# Autodesk Inventor assembly: 200-60-DIFFERENTIAL-BAR-01
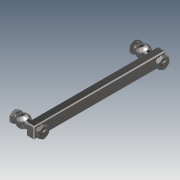
[picture p0: Inventor's stored thumbnail of the model, 180x180]
Saved by Autodesk Inventor 2018.2 (Build 222227000, 227)
## iProperties
Manager: feesmrt
Company: FRANCOR
Part Number: 200-60-DIFFERENTIAL-BAR-01
Project: Rescue Robot
Cost Center: -
Material: Generisch
Document SubType Name: Assembly
Designer: feesmrt
Engineer: feesmrt
Authority: feesmrt
Description: Differential Verbinder ASM
Stock Number: 200-60-DIFFERENTIAL-BAR-01
Subject: Rescue Robot
Author: feesmrt
Revision Number: 1
Title: Differential Verbinder ASM
## Documents named in this file (6)
- D:\Programmierung\FRANC0R\CAD\02-Rocker-Bogie-Robot\200-ROCKER-BOGIE\200-60-DIFFERENTIAL\200-60-DIFFERENTIAL-BAR-01.iam
- D:\Programmierung\FRANC0R\CAD\02-Rocker-Bogie-Robot\200-ROCKER-BOGIE\200-60-DIFFERENTIAL\200-60-DIFFERENTIAL-BAR-05.ipt
- D:\Programmierung\FRANC0R\CAD\02-Rocker-Bogie-Robot\200-ROCKER-BOGIE\200-60-DIFFERENTIAL\200-60-DIFFERENTIAL-BAR-04.ipt
- D:\Programmierung\FRANC0R\CAD\02-Rocker-Bogie-Robot\900-COMPONENTS\900-70-ANGLE-JOINTS\900-70-ANGLE-JOINT-DIN648-M8-2.ipt
- D:\Programmierung\FRANC0R\CAD\02-Rocker-Bogie-Robot\900-COMPONENTS\900-80-WASHERS\900-80-WASHERS-ISO8738-8.ipt
- D:\Programmierung\FRANC0R\CAD\02-Rocker-Bogie-Robot\900-COMPONENTS\900-41-NUTS\900-41-NUTS-ISO4035-M8.ipt
## Components (13 placed, 5 different names)
1. 200-60-DIFFERENTIAL-BAR-05:1 — Passend:1, Passend:2, Passend:4, Passend:13, Passend:16
2. 200-60-DIFFERENTIAL-BAR-04:1 — Passend:1, Passend:4, Passend:5, Passend:7, Passend:9, Passend:10, Passend:17, Passend:18
3. 200-60-DIFFERENTIAL-BAR-04:2 — Passend:2, Passend:6, Passend:8, Passend:11, Passend:12, Passend:23, Passend:24
4. 900-70-ANGLE-JOINT-DIN648-M8-2:1 — Passend:5, Passend:7, Passend:15
5. 900-70-ANGLE-JOINT-DIN648-M8-2:2 — Passend:6, Passend:8, Passend:14
6. 900-80-WASHERS-ISO8738-8:1 — Passend:12, Passend:13, Passend:21
7. 900-80-WASHERS-ISO8738-8:2 — Passend:11, Passend:14, Passend:22
8. 900-80-WASHERS-ISO8738-8:3 — Passend:9, Passend:16, Passend:20
9. 900-80-WASHERS-ISO8738-8:4 — Passend:10, Passend:15, Passend:19
10. 900-41-NUTS-ISO4035-M8:1 — Passend:21, Passend:24
11. 900-41-NUTS-ISO4035-M8:2 — Passend:22, Passend:23
12. 900-41-NUTS-ISO4035-M8:3 — Passend:17, Passend:20
13. 900-41-NUTS-ISO4035-M8:4 — Passend:18, Passend:19
## Relationships (23: Mate 23)
- Passend:1 [Mate]: 200-60-DIFFERENTIAL-BAR-05:1 ↔ 200-60-DIFFERENTIAL-BAR-04:1
- Passend:2 [Mate]: 200-60-DIFFERENTIAL-BAR-05:1 ↔ 200-60-DIFFERENTIAL-BAR-04:2
- Passend:4 [Mate]: 200-60-DIFFERENTIAL-BAR-05:1 ↔ 200-60-DIFFERENTIAL-BAR-04:1
- Passend:5 [Mate]: 200-60-DIFFERENTIAL-BAR-04:1 ↔ 900-70-ANGLE-JOINT-DIN648-M8-2:1
- Passend:6 [Mate]: 200-60-DIFFERENTIAL-BAR-04:2 ↔ 900-70-ANGLE-JOINT-DIN648-M8-2:2
- Passend:7 [Mate]: 200-60-DIFFERENTIAL-BAR-04:1 ↔ 900-70-ANGLE-JOINT-DIN648-M8-2:1
- Passend:8 [Mate]: 200-60-DIFFERENTIAL-BAR-04:2 ↔ 900-70-ANGLE-JOINT-DIN648-M8-2:2
- Passend:9 [Mate]: 200-60-DIFFERENTIAL-BAR-04:1 ↔ 900-80-WASHERS-ISO8738-8:3
- Passend:10 [Mate]: 200-60-DIFFERENTIAL-BAR-04:1 ↔ 900-80-WASHERS-ISO8738-8:4
- Passend:11 [Mate]: 200-60-DIFFERENTIAL-BAR-04:2 ↔ 900-80-WASHERS-ISO8738-8:2
- Passend:12 [Mate]: 200-60-DIFFERENTIAL-BAR-04:2 ↔ 900-80-WASHERS-ISO8738-8:1
- Passend:13 [Mate]: 200-60-DIFFERENTIAL-BAR-05:1 ↔ 900-80-WASHERS-ISO8738-8:1
- Passend:14 [Mate]: 900-70-ANGLE-JOINT-DIN648-M8-2:2 ↔ 900-80-WASHERS-ISO8738-8:2
- Passend:15 [Mate]: 900-70-ANGLE-JOINT-DIN648-M8-2:1 ↔ 900-80-WASHERS-ISO8738-8:4
- Passend:16 [Mate]: 200-60-DIFFERENTIAL-BAR-05:1 ↔ 900-80-WASHERS-ISO8738-8:3
- Passend:17 [Mate]: 200-60-DIFFERENTIAL-BAR-04:1 ↔ 900-41-NUTS-ISO4035-M8:3
- Passend:18 [Mate]: 200-60-DIFFERENTIAL-BAR-04:1 ↔ 900-41-NUTS-ISO4035-M8:4
- Passend:19 [Mate]: 900-80-WASHERS-ISO8738-8:4 ↔ 900-41-NUTS-ISO4035-M8:4
- Passend:20 [Mate]: 900-80-WASHERS-ISO8738-8:3 ↔ 900-41-NUTS-ISO4035-M8:3
- Passend:21 [Mate]: 900-80-WASHERS-ISO8738-8:1 ↔ 900-41-NUTS-ISO4035-M8:1
- Passend:22 [Mate]: 900-80-WASHERS-ISO8738-8:2 ↔ 900-41-NUTS-ISO4035-M8:2
- Passend:23 [Mate]: 200-60-DIFFERENTIAL-BAR-04:2 ↔ 900-41-NUTS-ISO4035-M8:2
- Passend:24 [Mate]: 200-60-DIFFERENTIAL-BAR-04:2 ↔ 900-41-NUTS-ISO4035-M8:1
